# Autodesk Inventor assembly: ultrasonic stuff
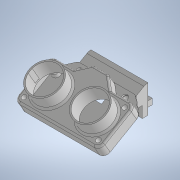
[picture p0: Inventor's stored thumbnail of the model, 180x180]
Saved by Autodesk Inventor 2022 (Build 260153000, 153)
## iProperties
Created: 2022-04-07
Part Number: ultrasonic stuff
Document SubType Name: Assembly
Designer: a-dubs
Author: a-dubs
## Documents named in this file (4)
- W:\My Drive\Coding and Projects\smart home\smart-deadbolt\3D Modelling\ultrasonic stuff.iam
- W:\My Drive\Coding and Projects\smart home\smart-deadbolt\3D Modelling\ultrasonic mount to deadbolt enclosure.ipt
- W:\My Drive\Coding and Projects\smart home\smart-deadbolt\3D Modelling\ultrasonic angled mount backing.ipt
- W:\My Drive\Coding and Projects\smart home\smart-deadbolt\3D Modelling\ultrasonic outer cover plate.ipt
## Components (3 placed, 3 different names)
1. ultrasonic mount to deadbolt enclosure:1 — Mate:1, Mate:2
2. ultrasonic angled mount backing:1 — Mate:1, Mate:2, Mate:3, Mate:4, Mate:5
3. ultrasonic outer cover plate:1 — Mate:3, Mate:4, Mate:5
## Relationships (5: Mate 5)
- Mate:1: ultrasonic mount to deadbolt enclosure:1 ↔ ultrasonic angled mount backing:1
- Mate:2: ultrasonic mount to deadbolt enclosure:1 ↔ ultrasonic angled mount backing:1
- Mate:3: ultrasonic angled mount backing:1 ↔ ultrasonic outer cover plate:1
- Mate:4: ultrasonic angled mount backing:1 ↔ ultrasonic outer cover plate:1
- Mate:5: ultrasonic angled mount backing:1 ↔ ultrasonic outer cover plate:1
